# Autodesk Inventor assembly: Сборка2
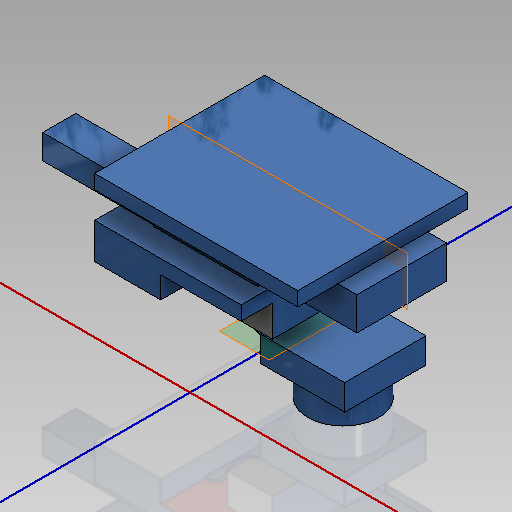
[picture p0: Inventor's stored thumbnail of the model, 512x512]
Saved by Autodesk Inventor 2021.2 (Build 252289000, 289)
## iProperties
Created: 2025-10-23
Part Number: Сборка2
Document SubType Name: Assembly
Designer: Захаров
Author: Захаров
## Documents named in this file (3)
- C:\Users\User\Documents\CaseARHead1\Сборка2.iam
- C:\Users\User\Documents\CaseARHead1\ЛЦМК0000002.00.00.00.00.03.ipt
- C:\Users\User\Documents\CaseARHead1\ЛЦМК0000002.00.00.00.00.04.ipt
## Components (2 placed, 2 different names)
1. ЛЦМК0000002.00.00.00.00.03:1 — Совмещение:1, Заподлицо:1, Заподлицо:2
2. ЛЦМК0000002.00.00.00.00.04 xiao cam:1 — Совмещение:1, Заподлицо:1, Заподлицо:2
## Relationships (3: Flush 2, Mate 1)
- Совмещение:1 [Mate]: ЛЦМК0000002.00.00.00.00.03:1 ↔ ЛЦМК0000002.00.00.00.00.04 xiao cam:1
- Заподлицо:1 [Flush]: ЛЦМК0000002.00.00.00.00.03:1 ↔ ЛЦМК0000002.00.00.00.00.04 xiao cam:1
- Заподлицо:2 [Flush]: ЛЦМК0000002.00.00.00.00.03:1 ↔ ЛЦМК0000002.00.00.00.00.04 xiao cam:1
